# Autodesk Inventor assembly: PCBA_estimation_20190215
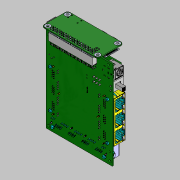
[picture p0: Inventor's stored thumbnail of the model, 180x180]
Saved by Autodesk Inventor 2020 (Build 240168000, 168)
## iProperties
Created: 2019-02-15
Part Number: PCBA_estimation_20190215
Document SubType Name: Assembly
Designer: Varga Daniel
Sending System: SolidWorks 2018
Last Author: david
Last Saved: 2019-02-15
Author: Varga Daniel
## Documents named in this file (8)
- C:\!_Dani\!_cloud\OneDrive\!_munka\Revolution\StructuralParts\Brain\Inventor imported\BRBETA-0618_Electronics assembly.iam
- C:\!_Dani\!_cloud\OneDrive\!_munka\Revolution\StructuralParts\Brain\Inventor imported\BRpcbA\carrier_board_2019-06-12.iam
- C:\!_Dani\!_cloud\OneDrive\!_munka\Revolution\StructuralParts\Brain\Inventor imported\BRled1\leds_board_2019-06-12.iam
- C:\!_Dani\!_cloud\OneDrive\!_munka\Revolution\StructuralParts\Brain\Inventor imported\PiZWA\PR(E,P)C020DAAN-RC.ipt
- C:\!_Dani\!_cloud\OneDrive\!_munka\Revolution\StructuralParts\Brain\Inventor imported\BRpcbA\SHR-05V-S-B.ipt
- C:\!_Dani\!_cloud\OneDrive\!_munka\Revolution\StructuralParts\Brain\Inventor imported\PiZWA\PiZWA.iam
- C:\!_Dani\!_cloud\OneDrive\!_munka\Revolution\StructuralParts\Brain\Inventor imported\BRBETA-0618_TF16gbA.ipt
- C:\!_Dani\!_cloud\OneDrive\!_munka\Revolution\StructuralParts\Brain\Inventor imported\BRBETA-0618_683866P_2000mAh.ipt
## Components (7 placed, 7 different names)
1. PiZWA:1 [sub-assembly] — Flush:9, Flush:10, Mate:2, Flush:11, Flush:12, Flush:13, Flush:14, Flush:15, Flush:16
2. RRRC_carrier_board:1 [sub-assembly] — Flush:14, Flush:15, Flush:16, Flush:17, Flush:18, Mate:3, Mate:4, Mate:5, Tangent:1, Tangent:2
3. RRRC_LED_board:1 [sub-assembly] — Flush:17, Flush:18, Mate:6
4. BRBETA-0618_TF16gbA:1 — Flush:11, Flush:12, Flush:13
5. BRBETA-0618_683866P_2000mAh:1 — Mate:6, Tangent:1, Tangent:2
6. PR(E,P)C020DAAN-RC:1 — Flush:9, Flush:10, Mate:2
7. SHR-05V-S-B:2 — Mate:3, Mate:4, Mate:5
## Relationships (17: Flush 10, Mate 5, Tangent 2)
- Flush:9 (-7.069 mm): PiZWA:1 ↔ PR(E,P)C020DAAN-RC:1
- Flush:10 (-0.883 mm): PiZWA:1 ↔ PR(E,P)C020DAAN-RC:1
- Mate:2: PiZWA:1 ↔ PR(E,P)C020DAAN-RC:1
- Flush:11 (-0.156 mm): PiZWA:1 ↔ BRBETA-0618_TF16gbA:1
- Flush:12 (-4.067 mm): PiZWA:1 ↔ BRBETA-0618_TF16gbA:1
- Flush:13 (0.506 mm): PiZWA:1 ↔ BRBETA-0618_TF16gbA:1
- Flush:14 (-3.54 mm): PiZWA:1 ↔ RRRC_carrier_board:1
- Flush:15 (-10.997 mm): PiZWA:1 ↔ RRRC_carrier_board:1
- Flush:16 (5.98 mm): PiZWA:1 ↔ RRRC_carrier_board:1
- Flush:17 (9.497 mm): RRRC_carrier_board:1 ↔ RRRC_LED_board:1
- Flush:18 (13.2 mm): RRRC_carrier_board:1 ↔ RRRC_LED_board:1
- Mate:3: RRRC_carrier_board:1 ↔ SHR-05V-S-B:2
- Mate:4: RRRC_carrier_board:1 ↔ SHR-05V-S-B:2
- Mate:5: RRRC_carrier_board:1 ↔ SHR-05V-S-B:2
- Mate:6: RRRC_LED_board:1 ↔ BRBETA-0618_683866P_2000mAh:1
- Tangent:1: RRRC_carrier_board:1 ↔ BRBETA-0618_683866P_2000mAh:1
- Tangent:2: RRRC_carrier_board:1 ↔ BRBETA-0618_683866P_2000mAh:1
